# Autodesk Inventor assembly: spherePlusSectC01
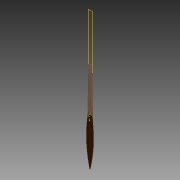
[picture p0: Inventor's stored thumbnail of the model, 180x180]
Saved by Autodesk Inventor 2013 (Build 170138000, 138)
## iProperties
Created: 2014-10-24
Part Number: spherePlusSectC01
Document SubType Name: Assembly
Designer: Nano
Author: Nano
## Documents named in this file (3)
- C:\Users\Nano\Documents\InventorByron\InventorMasterProject\octoBoto\spherePlusSectC01.iam
- C:\Users\Nano\Documents\InventorByron\InventorMasterProject\octoBoto\octoBotoStemSectC_v01.ipt
- C:\Users\Nano\Documents\InventorByron\InventorMasterProject\octoBoto\baseSphere01.ipt
## Components (2 placed, 2 different names)
1. octoBotoStemSectC_v01:1 — Mate:1, Mate:2, Mate:3
2. baseSphere01:1 — Mate:1, Mate:2, Mate:3
## Relationships (3: Mate 3)
- Mate:1: octoBotoStemSectC_v01:1 ↔ baseSphere01:1
- Mate:2: octoBotoStemSectC_v01:1 ↔ baseSphere01:1
- Mate:3 (-50.8 mm): octoBotoStemSectC_v01:1 ↔ baseSphere01:1
